# Autodesk Inventor assembly: Swing_Arm_06
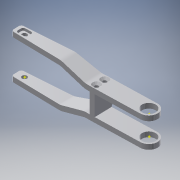
[picture p0: Inventor's stored thumbnail of the model, 180x180]
Saved by Autodesk Inventor 2016 (Build 200138000, 138)
## iProperties
Created: 2016-02-17
Part Number: Swing_Arm_06
Document SubType Name: Assembly
Designer: nils
Mass: 3573.9 g
Surface Area: 2154.53 cm^2
Volume: 1331.18 cm^3
Density: 2.68477 g/cm^3
Author: nils
## Documents named in this file (12)
- D:\bikair\Bikair_CAD-1\Source\Rear_Train\Swing_Arm_06.iam
- D:\bikair\Bikair_CAD-1\Source\Rear_Train\Profile_Straight_06.ipt
- D:\bikair\Bikair_CAD-1\Source\Rear_Train\Profile_Straight_MIR_06.ipt
- D:\bikair\Bikair_CAD-1\Source\Rear_Train\Profile_Middle_06.ipt
- D:\bikair\Bikair_CAD-1\Source\Rear_Train\Pin_01.ipt
- D:\bikair\Bikair_CAD-1\Source\Rear_Train\Dummy_Plug_01.ipt
- D:\bikair\Bikair_CAD-1\Source\Rear_Train\Swing_Arm_06\AIP\FEA\bp1hlflb4.fins
- D:\bikair\Bikair_CAD-1\Source\Rear_Train\Swing_Arm_06\AIP\FEA\bp1hlflb4.fsat
- D:\bikair\Bikair_CAD-1\Source\Rear_Train\Swing_Arm_06\AIP\FEA\bp1hlflb4.ftes
- D:\bikair\Bikair_CAD-1\Source\Rear_Train\Swing_Arm_06\AIP\FEA\bp1hlflb4.fwiz
- D:\bikair\Bikair_CAD-1\Source\Rear_Train\Swing_Arm_06\AIP\FEA\bp1hlflds.fmsh
- D:\bikair\Bikair_CAD-1\Source\Rear_Train\Swing_Arm_06\AIP\FEA\bp1hlfleo.fres
## Components (5 placed, 5 different names)
1. Profile_Straight_06:1 — Mate:1, Mate:2, Mate:3
2. Profile_Straight_MIR_06:1 — Mate:4, Mate:5, Mate:6
3. Profile_Middle_06:1 — Mate:1, Mate:2, Mate:3, Mate:4, Mate:5, Mate:6, Mate:7, Flush:1, Mate:9
4. Pin_01:1 — Mate:7, Flush:1, Mate:8
5. Dummy_Plug_01:1 — Mate:8, Mate:9
## Relationships (10: Mate 9, Flush 1)
- Mate:1: Profile_Straight_06:1 ↔ Profile_Middle_06:1
- Mate:2: Profile_Straight_06:1 ↔ Profile_Middle_06:1
- Mate:3: Profile_Straight_06:1 ↔ Profile_Middle_06:1
- Mate:4: Profile_Straight_MIR_06:1 ↔ Profile_Middle_06:1
- Mate:5: Profile_Straight_MIR_06:1 ↔ Profile_Middle_06:1
- Mate:6: Profile_Straight_MIR_06:1 ↔ Profile_Middle_06:1
- Mate:7: Profile_Middle_06:1 ↔ Pin_01:1
- Flush:1: Profile_Middle_06:1 ↔ Pin_01:1
- Mate:8: Pin_01:1 ↔ Dummy_Plug_01:1
- Mate:9 (5 mm): Profile_Middle_06:1 ↔ Dummy_Plug_01:1
## Named parameters: sa_0 = -10588.7, sa_1 = 399860, sa_2 = 1.935e-10, sa_3 = -10588.7, sa_4 = 399860, sa_5 = 3.045e-10
note: some values were not read from the file. Shown as the stored number, unit unknown: "sa_0", "sa_1", "sa_2", "sa_3", "sa_4", "sa_5".
